# Autodesk Inventor assembly: Tank tread link segment
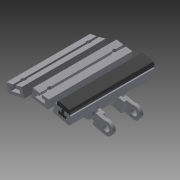
[picture p0: Inventor's stored thumbnail of the model, 180x180]
Saved by Autodesk Inventor 2015 (Build 190159000, 159)
## iProperties
Created: 2015-09-30
Part Number: Tank tread link segment
Document SubType Name: Assembly
Designer: alhohbein
Author: alhohbein
## Documents named in this file (3)
- U:\Tank tread link segment.iam
- U:\TETRIX_736468_TT_LINK_2012.ipt
- U:\Tank tread with rubber insert.iam
## Components (3 placed, 2 different names)
1. TETRIX_736468_TT_LINK_2012:1 — Insert:1, Insert:2
2. TETRIX_736468_TT_LINK_2012:2 — Insert:1
3. Tank tread with rubber insert:1 [sub-assembly] — Insert:2
## Relationships (2: Insert 2)
- Insert:1: TETRIX_736468_TT_LINK_2012:1 ↔ TETRIX_736468_TT_LINK_2012:2
- Insert:2: TETRIX_736468_TT_LINK_2012:1 ↔ Tank tread with rubber insert:1
